# Autodesk Inventor assembly: 24T nanotube cluster
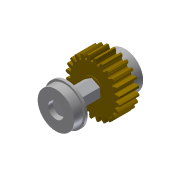
[picture p0: Inventor's stored thumbnail of the model, 180x180]
Saved by Autodesk Inventor 2013 (Build 170138000, 138)
## iProperties
Created: 2013-09-01
Part Number: 24T nanotube cluster
Document SubType Name: Assembly
Designer: Nemo
Author: Nemo
## Documents named in this file (4)
- H:\Nemo\Documents\Robotics\COTS Parts\Gearboxes\Components\24T nanotube cluster.iam
- H:\Nemo\Documents\Robotics\COTS Parts\Bearings - VexPro\Flanged Bearing - 0.375in Round ID x 0.875in OD.ipt
- H:\Nemo\Documents\Robotics\COTS Parts\Gearboxes\Components\VexPro Double Reduction Components\VexBox cluster shaft.ipt
- H:\Nemo\Documents\Robotics\COTS Parts\Gears - VexPro\Gear 20dp 375hex 24T Vex.ipt
## Components (4 placed, 3 different names)
1. Flanged Bearing - 0.375in Round ID x 0.875in OD:1 — Mate:2
2. VexBox cluster shaft:1 — Mate:1, Mate:4, Angle:1, Mate:5
3. Flanged Bearing - 0.375in Round ID x 0.875in OD:2 — Mate:1, Mate:2, Mate:4, Mate:6
4. Gear 20dp 375hex 24T Vex:1 — Angle:1, Mate:5, Mate:6
## Relationships (6: Mate 5, Angle 1)
- Mate:1: VexBox cluster shaft:1 ↔ Flanged Bearing - 0.375in Round ID x 0.875in OD:2
- Mate:2 (-31.75 mm): Flanged Bearing - 0.375in Round ID x 0.875in OD:1 ↔ Flanged Bearing - 0.375in Round ID x 0.875in OD:2
- Mate:4 (0.254 mm): VexBox cluster shaft:1 ↔ Flanged Bearing - 0.375in Round ID x 0.875in OD:2
- Angle:1 (0 deg): VexBox cluster shaft:1 ↔ Gear 20dp 375hex 24T Vex:1
- Mate:5: VexBox cluster shaft:1 ↔ Gear 20dp 375hex 24T Vex:1
- Mate:6 (0.254 mm): Flanged Bearing - 0.375in Round ID x 0.875in OD:2 ↔ Gear 20dp 375hex 24T Vex:1
